# Autodesk Inventor assembly: Baugruppe1
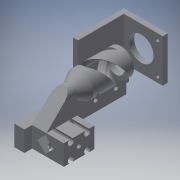
[picture p0: Inventor's stored thumbnail of the model, 180x180]
Saved by Autodesk Inventor 2019 (Build 230136000, 136)
## iProperties
Created: 2021-06-02
Part Number: Baugruppe1
Material: Generisch
Document SubType Name: Assembly
Designer: Bergi
Author: Bergi
## Documents named in this file (5)
- C:\Users\Bergi\Desktop\3D Sketches\Bleistift_Plotter\Baugruppe1.iam
- C:\Users\Bergi\Desktop\3D Sketches\Bleistift_Plotter\Spirale_Korb.ipt
- C:\Users\Bergi\Desktop\3D Sketches\Bleistift_Plotter\Schlitten_neu.ipt
- C:\Users\Bergi\Desktop\3D Sketches\Bleistift_Plotter\Backplate.ipt
- C:\Users\Bergi\Desktop\3D Sketches\Bleistift_Plotter\Linear_rail.ipt
## Components (4 placed, 4 different names)
1. Spirale_Korb:1 — Passend:3, Passend:4, Winkel:1
2. Schlitten_neu:1 — Passend:1, Passend:2, Passend:3, Passend:4
3. Backplate:1 — Passend:5, Winkel:1
4. Linear_rail:1 — Passend:1, Passend:2, Passend:5
## Relationships (6: Mate 5, Angle 1)
- Passend:1 [Mate]: Schlitten_neu:1 ↔ Linear_rail:1
- Passend:2 [Mate]: Schlitten_neu:1 ↔ Linear_rail:1
- Passend:3 [Mate]: Spirale_Korb:1 ↔ Schlitten_neu:1
- Passend:4 [Mate]: Spirale_Korb:1 ↔ Schlitten_neu:1
- Passend:5 [Mate]: Backplate:1 ↔ Linear_rail:1
- Winkel:1 [Angle] (180 deg): Spirale_Korb:1 ↔ Backplate:1
